# Autodesk Inventor assembly: Assembly7
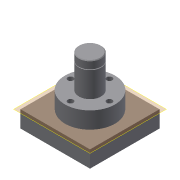
[picture p0: Inventor's stored thumbnail of the model, 180x180]
Saved by Autodesk Inventor 2017 (Build 210142000, 142)
## iProperties
Created: 2016-07-28
Part Number: Assembly7
Document SubType Name: Assembly
Designer: Tutorial Books
Author: Tutorial Books
## Documents named in this file (4)
- C:\Users\anand\Documents\Inventor\Autodesk Inventor 2017 Learn by doing\C07_tut1\Assembly7.iam
- C:\Users\anand\Documents\Inventor\Autodesk Inventor 2017 Learn by doing\C07_tut1\Base.ipt
- C:\Users\anand\Documents\Inventor\Autodesk Inventor 2017 Learn by doing\C07_tut1\Spacer.ipt
- C:\Users\anand\Documents\Inventor\Autodesk Inventor 2017 Learn by doing\C07_tut1\Shoulder Screw.ipt
## Components (3 placed, 3 different names)
1. Base:1 — Flush:1, Flush:2, Flush:3, Flush:4
2. Spacer:1 — Flush:2, Flush:3
3. Shoulder Screw:1 — Flush:4
## Relationships (4: Flush 4)
- Flush:1: Base:1
- Flush:2: Base:1 ↔ Spacer:1
- Flush:3: Base:1 ↔ Spacer:1
- Flush:4: Base:1 ↔ Shoulder Screw:1
